# Autodesk Inventor assembly: wheel4
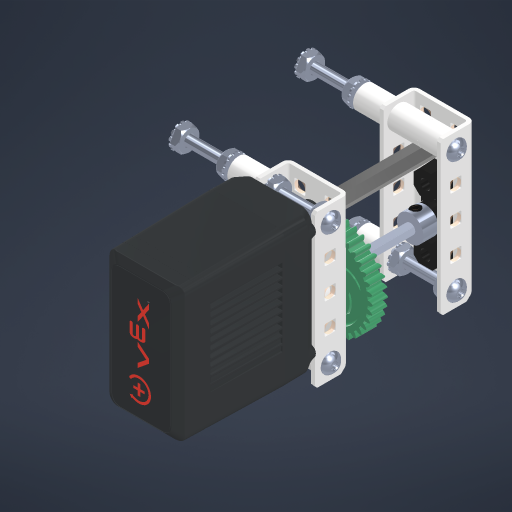
[picture p0: Inventor's stored thumbnail of the model, 512x512]
Saved by Autodesk Inventor 2024 (Build 280153000, 153)
## iProperties
Created: 2023-08-09
Part Number: wheel4
Document SubType Name: Assembly
Designer: macbook
Author: macbook
## Documents named in this file (24)
- \\Mac\Home\Desktop\code\7899V-VRC-OVER-UNDER\Cad\VEX-CAD-Inventor-1.4.0\Assembly\v0.2\wheel4.iam
- \\Mac\Home\Desktop\code\7899V-VRC-OVER-UNDER\Cad\VEX-CAD-Inventor-1.4.0\Motion\Gears\LS 36T Gear.ipt
- \\Mac\Home\Desktop\code\7899V-VRC-OVER-UNDER\Cad\VEX-CAD-Inventor-1.4.0\Motion\Shaft LS\Bearing Flat.ipt
- \\Mac\Home\Desktop\code\7899V-VRC-OVER-UNDER\Cad\VEX-CAD-Inventor-1.4.0\Motion\Shaft LS\Shaft LS.ipt
- \\Mac\Home\Desktop\code\7899V-VRC-OVER-UNDER\Cad\VEX-CAD-Inventor-1.4.0\Motion\Shaft LS\Shaft Collar Metal\Shaft Collar Set Screw.iam
- \\Mac\Home\Desktop\code\7899V-VRC-OVER-UNDER\Cad\VEX-CAD-Inventor-1.4.0\Motion\Shaft LS\Shaft Collar Metal.iam
- \\Mac\Home\Desktop\code\7899V-VRC-OVER-UNDER\Cad\VEX-CAD-Inventor-1.4.0\Electronics\Motors with Screws\AluM-StarS.iam
- \\Mac\Home\Desktop\code\7899V-VRC-OVER-UNDER\Cad\VEX-CAD-Inventor-1.4.0\Electronics\Motors with Screws.iam
- \\Mac\Home\Desktop\code\7899V-VRC-OVER-UNDER\Cad\VEX-CAD-Inventor-1.4.0\Motion\Spacers\Spacer Nylon .500 OD\NSpacer White .500 OD x .375.ipt
- \\Mac\Home\Desktop\code\7899V-VRC-OVER-UNDER\Cad\VEX-CAD-Inventor-1.4.0\Motion\Spacers\Spacer Nylon .500 OD.ipt
- \\Mac\Home\Desktop\code\7899V-VRC-OVER-UNDER\Cad\VEX-CAD-Inventor-1.4.0\Structure\Hardware\Screw Steel - Star.ipt
- \\Mac\Home\Desktop\code\7899V-VRC-OVER-UNDER\Cad\VEX-CAD-Inventor-1.4.0\Structure\C Channel\Aluminum 1x2x1\Alu C 1x2x1x5.ipt
- \\Mac\Home\Desktop\code\7899V-VRC-OVER-UNDER\Cad\VEX-CAD-Inventor-1.4.0\Structure\Hardware\Nut Keps.ipt
- \\Mac\Home\Desktop\code\7899V-VRC-OVER-UNDER\Cad\VEX-CAD-Inventor-1.4.0\Motion\Spacers\Spacer Nylon .313 OD\NSpacer .313 OD x .375.ipt
- \\Mac\Home\Desktop\code\7899V-VRC-OVER-UNDER\Cad\VEX-CAD-Inventor-1.4.0\Motion\Spacers\Spacer Nylon .313 OD.ipt
- \\Mac\Home\Desktop\code\7899V-VRC-OVER-UNDER\Cad\VEX-CAD-Inventor-1.4.0\Motion\Spacers\Spacer Nylon .313 OD\NSpacer .313 OD x .500.ipt
- \\Mac\Home\Desktop\code\7899V-VRC-OVER-UNDER\Cad\VEX-CAD-Inventor-1.4.0\Structure\Hardware\Screw Steel - Star\SScrew Star Smooth 2.500.ipt
- \\Mac\Home\Desktop\code\7899V-VRC-OVER-UNDER\Cad\VEX-CAD-Inventor-1.4.0\Structure\Hardware\Screw Steel - Star\SScrew Star Smooth 1.750.ipt
- \\Mac\Home\Desktop\code\7899V-VRC-OVER-UNDER\Cad\VEX-CAD-Inventor-1.4.0\Structure\Hardware\Nut Thin Nylock.ipt
- \\Mac\Home\Desktop\code\7899V-VRC-OVER-UNDER\Cad\VEX-CAD-Inventor-1.4.0\Structure\Standoff.ipt
- \\Mac\Home\Desktop\code\7899V-VRC-OVER-UNDER\Cad\VEX-CAD-Inventor-1.4.0\Structure\Standoff\Standoff 2.00.ipt
- \\Mac\Home\Desktop\code\7899V-VRC-OVER-UNDER\Cad\VEX-CAD-Inventor-1.4.0\Motion\Spacers\Washer Teflon\TWasher .375 OD x .03125.ipt
- \\Mac\Home\Desktop\code\7899V-VRC-OVER-UNDER\Cad\VEX-CAD-Inventor-1.4.0\Motion\Spacers\Washer Teflon.ipt
- \\Mac\Home\Desktop\code\7899V-VRC-OVER-UNDER\Cad\VEX-CAD-Inventor-1.4.0\Motion\Shaft LS\Shaft LS\Shaft LS 3.0.ipt
## Components (34 placed, 15 different names)
1. LS 36T Gear:1
2. Bearing Flat:1 — Insert:10
3. Shaft LS 3.0:1 — Mate:1
4. Shaft Collar Set Screw:1 [sub-assembly]
5. Shaft Collar Set Screw:2 [sub-assembly]
6. AluM-StarS:1 [sub-assembly] — Mate:1
7. NSpacer White .500 OD x .375:1 — Insert:12
8. TWasher .375 OD x .03125:1
9. Alu C 1x2x1x5:1 — Insert:12, Insert:13, Insert:16, Insert:17, Insert:21, Insert:23, Insert:24, Insert:29, Insert:34
10. Alu C 1x2x1x5:2 — Insert:10, Insert:13, Insert:14, Insert:15, Insert:20, Insert:22, Insert:25, Insert:26, Insert:35, Insert:38
11. Nut Keps:1 — Insert:14
12. Nut Keps:3 — Insert:15
13. Nut Keps:4 — Insert:16
14. Nut Keps:5 — Insert:17
15. NSpacer .313 OD x .375:1 — Insert:18
16. NSpacer .313 OD x .500:2 — Insert:18, Insert:20
17. NSpacer .313 OD x .375:3
18. NSpacer .313 OD x .500:4 — Insert:21
19. NSpacer .313 OD x .500:5 — Insert:22, Insert:27
20. NSpacer .313 OD x .500:6 — Insert:23, Insert:36
21. NSpacer .313 OD x .500:7 — Insert:25, Insert:37
22. NSpacer .313 OD x .500:8 — Insert:24, Insert:30
23. SScrew Star Smooth 2.500:1 — Insert:26
24. Nut Keps:6 — Insert:27, Insert:28
25. Nut Keps:7 — Insert:28
26. SScrew Star Smooth 1.750:2 — Insert:29
27. Nut Thin Nylock:1 — Insert:30
28. Nut Keps:8 — Insert:36
29. Nut Keps:9
30. SScrew Star Smooth 2.500:4 — Insert:35
31. SScrew Star Smooth 2.500:5 — Insert:34
32. Nut Keps:12 — Insert:37
33. Nut Keps:13
34. Standoff 2.00:1 — Insert:38
## Relationships (35: Insert 32, CylindricalJoint 2, Mate 1)
- [Insert]: LS 36T Gear:1 ↔ TWasher .375 OD x .03125:1
- [Insert]: LS 36T Gear:1 ↔ Shaft Collar Set Screw:2
- [Insert] (1.5875 mm): NSpacer White .500 OD x .375:1 ↔ TWasher .375 OD x .03125:1
- [Insert] (46.8313 mm): Bearing Flat:1 ↔ AluM-StarS:1
- [Insert]: Bearing Flat:1 ↔ Shaft Collar Set Screw:1
- [CylindricalJoint]: Bearing Flat:1 ↔ Shaft LS 3.0:1
- [CylindricalJoint]: Shaft LS 3.0:1 ↔ Shaft Collar Set Screw:2
- Insert:10: Bearing Flat:1 ↔ Alu C 1x2x1x5:2
- Insert:12: NSpacer White .500 OD x .375:1 ↔ Alu C 1x2x1x5:1
- Insert:13 (50.8 mm): Alu C 1x2x1x5:1 ↔ Alu C 1x2x1x5:2
- Insert:14: Alu C 1x2x1x5:2 ↔ Nut Keps:1
- Insert:15: Alu C 1x2x1x5:2 ↔ Nut Keps:3
- Insert:16: Alu C 1x2x1x5:1 ↔ Nut Keps:4
- Insert:17: Alu C 1x2x1x5:1 ↔ Nut Keps:5
- Insert:18: NSpacer .313 OD x .375:1 ↔ NSpacer .313 OD x .500:2
- [Insert]: NSpacer .313 OD x .375:3 ↔ NSpacer .313 OD x .500:4
- Insert:20: Alu C 1x2x1x5:2 ↔ NSpacer .313 OD x .500:2
- Insert:21: Alu C 1x2x1x5:1 ↔ NSpacer .313 OD x .500:4
- Insert:22: Alu C 1x2x1x5:2 ↔ NSpacer .313 OD x .500:5
- Insert:23: Alu C 1x2x1x5:1 ↔ NSpacer .313 OD x .500:6
- Insert:24: Alu C 1x2x1x5:1 ↔ NSpacer .313 OD x .500:8
- Insert:25: Alu C 1x2x1x5:2 ↔ NSpacer .313 OD x .500:7
- Insert:26: Alu C 1x2x1x5:2 ↔ SScrew Star Smooth 2.500:1
- Insert:27 (1.5875 mm): NSpacer .313 OD x .500:5 ↔ Nut Keps:6
- Insert:28 (15.24 mm): Nut Keps:6 ↔ Nut Keps:7
- Insert:29: Alu C 1x2x1x5:1 ↔ SScrew Star Smooth 1.750:2
- Insert:30 (1.5875 mm): NSpacer .313 OD x .500:8 ↔ Nut Thin Nylock:1
- [Insert] (15.24 mm): Nut Keps:8 ↔ Nut Keps:9
- [Insert] (15.24 mm): Nut Keps:12 ↔ Nut Keps:13
- Insert:34: Alu C 1x2x1x5:1 ↔ SScrew Star Smooth 2.500:5
- Insert:35: Alu C 1x2x1x5:2 ↔ SScrew Star Smooth 2.500:4
- Insert:36 (1.5875 mm): NSpacer .313 OD x .500:6 ↔ Nut Keps:8
- Insert:37 (1.5875 mm): NSpacer .313 OD x .500:7 ↔ Nut Keps:12
- Mate:1: Shaft LS 3.0:1 ↔ AluM-StarS:1
- Insert:38: Alu C 1x2x1x5:2 ↔ Standoff 2.00:1
## Named parameters: d3_d9 = 46.83125 mm, d4_d11 = 0 mm, d10_d13 = 86.543877 deg, d33_d32 = 0 mm, d45_d42 = 15.24 mm, d47_d42 = 15.24 mm
